# Autodesk Inventor assembly: Picker with BBM
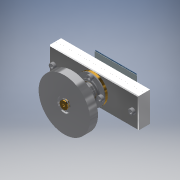
[picture p0: Inventor's stored thumbnail of the model, 180x180]
Saved by Autodesk Inventor 2019.4 (Build 234330000, 330)
## iProperties
Created: 2021-01-15
Part Number: Picker with BBM
Document SubType Name: Assembly
Designer: caleb
Author: caleb
## Documents named in this file (3)
- C:\Users\cfang\Desktop\nebraska-silicon-lab\CAD\ETL\Module Assembly\Picker with BBM.iam
- C:\Users\cfang\Desktop\nebraska-silicon-lab\CAD\ETL\Module Assembly\Picker Tool\Picker Tool.iam
- C:\Users\cfang\Desktop\nebraska-silicon-lab\CAD\ETL\Module Assembly\BBM Staging Plate\Bare Bump-Bonded Module.iam
## Components (2 placed, 2 different names)
1. Picker Tool:1 [sub-assembly] — Mate:1, Angle:1
2. Bare Bump-Bonded Module:1 [sub-assembly] — Mate:1, Angle:1
## Relationships (2: Mate 1, Angle 1)
- Mate:1: Picker Tool:1 ↔ Bare Bump-Bonded Module:1
- Angle:1 (0 deg): Picker Tool:1 ↔ Bare Bump-Bonded Module:1
